# Autodesk Inventor assembly: Kanawa Tsugi
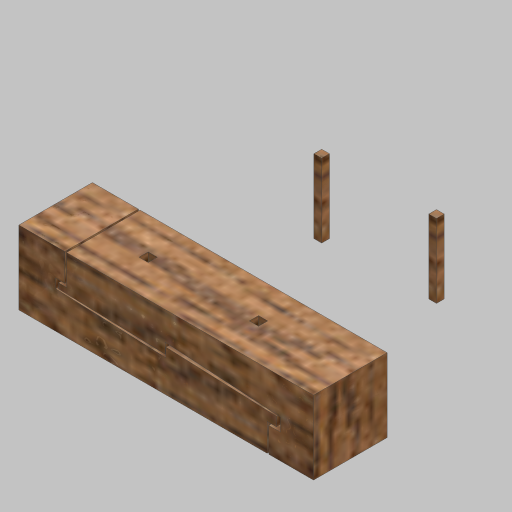
[picture p0: Inventor's stored thumbnail of the model, 512x512]
Saved by Autodesk Inventor 2023 (Build 270158000, 158)
## iProperties
Created: 2026-07-03
Part Number: Kanawa Tsugi
Document SubType Name: Assembly
Designer: MARTIN MAESTRE
Author: MARTIN MAESTRE
## Documents named in this file (4)
- C:\Users\MARTIN MAESTRE\OneDrive - Universidad de los Andes\POSTGRADO\202610\MAESTRIA\PROBLEMA ESPECIAL\CADS_TOLERANCIAS\Repositorio\Kanawa Tsugi\Kanawa Tsugi.iam
- C:\Users\MARTIN MAESTRE\OneDrive - Universidad de los Andes\POSTGRADO\202610\MAESTRIA\PROBLEMA ESPECIAL\CADS_TOLERANCIAS\Repositorio\Kanawa Tsugi\Part_Female.ipt
- C:\Users\MARTIN MAESTRE\OneDrive - Universidad de los Andes\POSTGRADO\202610\MAESTRIA\PROBLEMA ESPECIAL\CADS_TOLERANCIAS\Repositorio\Kanawa Tsugi\Part_Male.ipt
- C:\Users\MARTIN MAESTRE\OneDrive - Universidad de los Andes\POSTGRADO\202610\MAESTRIA\PROBLEMA ESPECIAL\CADS_TOLERANCIAS\Repositorio\Kanawa Tsugi\Pins.ipt
## Components (4 placed, 3 different names)
1. Part_Female:1 — Coincidencia:1, Nivelación:1, Coincidencia:2, Nivelación:2, Nivelación:3
2. Part_Male:1 — Nivelación:2, Nivelación:3
3. Pins:1
4. Pins:2
## Relationships (5: Flush 3, Mate 2)
- Coincidencia:1 [Mate]: Part_Female:1
- Nivelación:1 [Flush]: Part_Female:1
- Coincidencia:2 [Mate]: Part_Female:1
- Nivelación:2 [Flush]: Part_Female:1 ↔ Part_Male:1
- Nivelación:3 [Flush]: Part_Female:1 ↔ Part_Male:1
